# Autodesk Inventor assembly: M - hook block
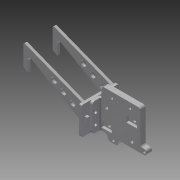
[picture p0: Inventor's stored thumbnail of the model, 180x180]
Saved by Autodesk Inventor 2013 (Build 170138000, 138)
## iProperties
Created: 2013-01-27
Part Number: M - hook block
Document SubType Name: Assembly
Designer: Arpan
Mass: 1657.38 g
Surface Area: 867.213 cm^2
Volume: 211.132 cm^3
Density: 7.85 g/cm^3
Author: Arpan
## Documents named in this file (5)
- C:\Users\Moses\Documents\Inventor\M - hook block.iam
- C:\Users\Moses\Documents\GitHub\frc2013CAD\Cimber actual\hook mount plate 2.ipt
- C:\Users\Moses\Documents\GitHub\frc2013CAD\Cimber actual\hook mount plate.ipt
- C:\Users\Moses\Documents\GitHub\frc2013CAD\Cimber actual\hook faceplate.ipt
- C:\Users\Moses\Documents\GitHub\frc2013CAD\Cimber actual\hook.ipt
## Components (5 placed, 4 different names)
1. hook mount plate 2:1 — Mate:5, Flush:2, Flush:3, Flush:5, Mate:6, Mate:13
2. hook mount plate:1 — Mate:5, Flush:2, Flush:3, Flush:4, Mate:13
3. hook faceplate:1 — Mate:6, Flush:4, Flush:5, Mate:7, Mate:8, Mate:9, Mate:10, Mate:11, Mate:12
4. hook:1 — Mate:10, Mate:11, Mate:12
5. hook:2 — Mate:7, Mate:8, Mate:9
## Relationships (13: Mate 9, Flush 4)
- Mate:5: hook mount plate 2:1 ↔ hook mount plate:1
- Flush:2: hook mount plate 2:1 ↔ hook mount plate:1
- Flush:3: hook mount plate 2:1 ↔ hook mount plate:1
- Mate:6: hook mount plate 2:1 ↔ hook faceplate:1
- Flush:4 (-38.1 mm): hook mount plate:1 ↔ hook faceplate:1
- Flush:5: hook mount plate 2:1 ↔ hook faceplate:1
- Mate:7: hook faceplate:1 ↔ hook:2
- Mate:8: hook faceplate:1 ↔ hook:2
- Mate:9: hook faceplate:1 ↔ hook:2
- Mate:10: hook faceplate:1 ↔ hook:1
- Mate:11: hook faceplate:1 ↔ hook:1
- Mate:12: hook faceplate:1 ↔ hook:1
- Mate:13: hook mount plate 2:1 ↔ hook mount plate:1
